# Autodesk Inventor assembly: Core
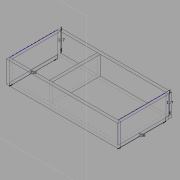
[picture p0: Inventor's stored thumbnail of the model, 180x180]
Saved by Autodesk Inventor 2022 (Build 260153000, 153)
## iProperties
Created: 2022-04-08
Part Number: Core
Document SubType Name: Assembly
Designer: Kalugin_a
Author: Kalugin_a
## Documents named in this file (8)
- C:\Users\A\Documents\GitHub\Melas-DIII-base\Workspace\BoordyaBeatBox\Core.iam
- C:\Users\A\Documents\GitHub\Melas-DIII-base\Workspace\BoordyaBeatBox\Front_L.ipt
- C:\Users\A\Documents\GitHub\Melas-DIII-base\Workspace\BoordyaBeatBox\Front1.ipt
- C:\Users\A\Documents\GitHub\Melas-DIII-base\Workspace\BoordyaBeatBox\Top.ipt
- C:\Users\A\Documents\GitHub\Melas-DIII-base\Workspace\BoordyaBeatBox\side.ipt
- C:\Users\A\Documents\GitHub\Melas-DIII-base\Workspace\BoordyaBeatBox\bottom.ipt
- C:\Users\A\Documents\GitHub\Melas-DIII-base\Workspace\DIII\внутр.ipt
- C:\Users\A\Documents\GitHub\Melas-DIII-base\Workspace\DIII\задник.ipt
## Components (8 placed, 7 different names)
1. Front_L:1 — Совмещение:3, Совмещение:5, Совмещение:7, Совмещение:11, Совмещение:12, Совмещение:13
2. Front1:1 — Совмещение:11, Совмещение:12
3. Top:1 — Совмещение:3, Совмещение:6, Совмещение:17
4. side:1 — Совмещение:5, Совмещение:6, Совмещение:8, Совмещение:16
5. bottom:1 — Совмещение:7, Совмещение:8, Совмещение:14, Совмещение:15
6. side:2 — Совмещение:13, Совмещение:14
7. внутр:1 — Совмещение:15
8. задник:1 — Совмещение:16, Совмещение:17
## Relationships (12: Mate 12)
- Совмещение:3 [Mate]: Front_L:1 ↔ Top:1
- Совмещение:5 [Mate]: Front_L:1 ↔ side:1
- Совмещение:6 [Mate]: Top:1 ↔ side:1
- Совмещение:7 [Mate]: Front_L:1 ↔ bottom:1
- Совмещение:8 [Mate]: side:1 ↔ bottom:1
- Совмещение:11 [Mate]: Front_L:1 ↔ Front1:1
- Совмещение:12 [Mate]: Front_L:1 ↔ Front1:1
- Совмещение:13 [Mate]: Front_L:1 ↔ side:2
- Совмещение:14 [Mate]: bottom:1 ↔ side:2
- Совмещение:15 [Mate]: bottom:1 ↔ внутр:1
- Совмещение:16 [Mate]: side:1 ↔ задник:1
- Совмещение:17 [Mate]: Top:1 ↔ задник:1
